# Autodesk Inventor assembly: bearing_holder
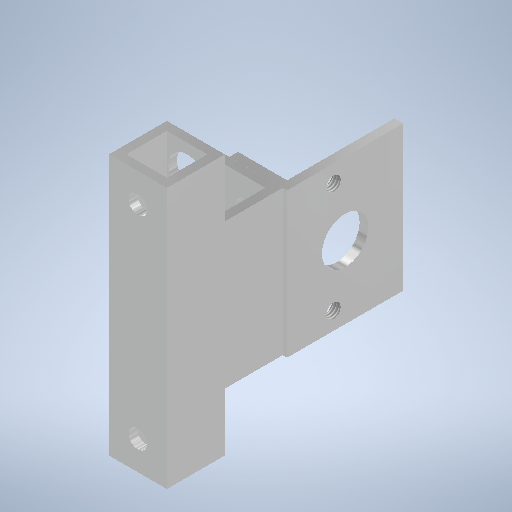
[picture p0: Inventor's stored thumbnail of the model, 512x512]
Saved by Autodesk Inventor 2025 (Build 290162000, 162)
## iProperties
Created: 2024-04-25
Part Number: bearing_holder
Document SubType Name: Assembly
Designer: rader
Author: rader
## Documents named in this file (4)
- C:\Users\rader\Documents\rp\bearing_holder.iam
- C:\Users\rader\Documents\rp\bearing_base.ipt
- C:\Users\rader\Documents\rp\bearing_holder.ipt
- C:\Users\rader\Documents\rp\bearing_standoff.ipt
## Components (3 placed, 3 different names)
1. bearing_base:1 — Vložit:2, Vložit:4
2. bearing_holder:1 — Proti sobě:1, Vložit:1, Vložit:3
3. bearing_standoff:1 — Proti sobě:1, Vložit:1, Vložit:2, Vložit:3, Vložit:4
## Relationships (5: Insert 4, Mate 1)
- Proti sobě:1 [Mate]: bearing_holder:1 ↔ bearing_standoff:1
- Vložit:1 [Insert]: bearing_holder:1 ↔ bearing_standoff:1
- Vložit:2 [Insert]: bearing_base:1 ↔ bearing_standoff:1
- Vložit:3 [Insert]: bearing_holder:1 ↔ bearing_standoff:1
- Vložit:4 [Insert]: bearing_base:1 ↔ bearing_standoff:1
